# Autodesk Inventor assembly: Bike_Drive
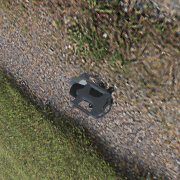
[picture p0: Inventor's stored thumbnail of the model, 180x180]
Saved by Autodesk Inventor 2016 (Build 200138000, 138)
## iProperties
Created: 2015-05-13
Part Number: Bike_Drive
Document SubType Name: Assembly
Designer: Yann
Author: Yann
## Documents named in this file (11)
- C:\Users\Yann\Documents\GitHub\BIKAIR_CAD\Source\Bike_Drive\Bike_Drive.iam
- C:\Users\Yann\Documents\GitHub\BIKAIR_CAD\Source\Bike_Drive\DEFAULT.ipt
- C:\Users\Yann\Documents\GitHub\BIKAIR_CAD\Source\Bike_Drive\DEFAULT_1.ipt
- C:\Users\Yann\Documents\GitHub\BIKAIR_CAD\Source\Bike_Drive\DEFAULT_2.ipt
- C:\Users\Yann\Documents\GitHub\BIKAIR_CAD\Source\Bike_Drive\DEFAULT_3.ipt
- C:\Users\Yann\Documents\GitHub\BIKAIR_CAD\Source\Bike_Drive\DEFAULT_4.ipt
- C:\Users\Yann\Documents\GitHub\BIKAIR_CAD\Source\Bike_Drive\DEFAULT_5.ipt
- C:\Users\Yann\Documents\GitHub\BIKAIR_CAD\Source\Bike_Drive\DEFAULT_6.ipt
- C:\Users\Yann\Documents\GitHub\BIKAIR_CAD\Source\Bike_Drive\DEFAULT_7.ipt
- C:\Users\Yann\Documents\GitHub\BIKAIR_CAD\Source\Bike_Drive\DEFAULT.iam
- C:\Users\Yann\Documents\GitHub\BIKAIR_CAD\Source\Bike_Drive\DEFAULT_1.iam
## Components (22 placed, 8 different names)
1. DEFAULT
2. DEFAULT:1
3. DEFAULT_1
4. DEFAULT_2
5. DEFAULT_3 — Rotational:2
6. DEFAULT_4
7. DEFAULT_5
8. DEFAULT_6
9. DEFAULT_6:1
10. DEFAULT_6:2
11. DEFAULT_6:3
12. DEFAULT_6:4
13. DEFAULT_6:5
14. DEFAULT_6:6
15. DEFAULT_6:7
16. DEFAULT_7
17. DEFAULT_7:1
18. DEFAULT_7:2
19. DEFAULT_7:3
20. DEFAULT:2 [sub-assembly] — Rotational:1
21. DEFAULT_1:1 [sub-assembly] — Rotational:2
22. DEFAULT_1:2 [sub-assembly] — Rotational:1
## Relationships (2: RevoluteJoint 2)
- Rotational:1 [RevoluteJoint]: DEFAULT:2 ↔ DEFAULT_1:2
- Rotational:2 [RevoluteJoint]: DEFAULT_3 ↔ DEFAULT_1:1
